# Autodesk Inventor assembly: Assembly1
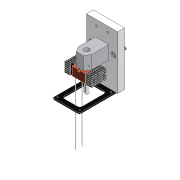
[picture p0: Inventor's stored thumbnail of the model, 180x180]
Saved by Autodesk Inventor 2022.4 (Build 264492000, 492)
## iProperties
Category: -
Company: Universiteit van Amsterdam
Created: 2023-08-21
Part Number: Assembly1
Document SubType Name: Assembly
Designer: RbSrWorkstation1
User Status: Work in Progress
Author: RbSrWorkstation1
Revision Number: A
## Documents named in this file (18)
- D:\VaultLocalWorkingFolder\UvA_MT\Projects\2023\23-0064 Laser diode holder Prem\20_3D-Models\23-0064  Laser diode collimator holder.iam
- D:\VaultLocalWorkingFolder\UvA_MT\Projects\2023\23-0064 Laser diode holder Prem\20_3D-Models\K+S 20C-A4.5-07.ipt
- D:\VaultLocalWorkingFolder\UvA_MT\Projects\2023\23-0064 Laser diode holder Prem\20_3D-Models\23-0064 Diode holder.ipt
- D:\VaultLocalWorkingFolder\UvA_MT\Projects\2023\23-0064 Laser diode holder Prem\20_3D-Models\23-0064 Cooling block.ipt
- D:\VaultLocalWorkingFolder\UvA_MT\Projects\2023\23-0064 Laser diode holder Prem\20_3D-Models\TECF1S.ipt
- D:\VaultLocalWorkingFolder\UvA_MT\Projects\2023\23-0064 Laser diode holder Prem\20_3D-Models\ick_bga_33x33x14.ipt
- D:\VaultLocalWorkingFolder\UvA_MT\Projects\2023\23-0064 Laser diode holder Prem\20_3D-Models\23-0064 Base plate.ipt
- D:\VaultLocalWorkingFolder\UvA_MT\Projects\2023\23-0064 Laser diode holder Prem\20_3D-Models\23-0064  PCB plate.ipt
- D:\VaultLocalWorkingFolder\UvA_MT\Content_Center_Files\en-US\DIN 912\DIN 912 - M5 x 0.8 x 10 x 8.ipt
- D:\VaultLocalWorkingFolder\UvA_MT\Content_Center_Files\en-US\DIN 912\DIN 912 - M6 x 1 x 20 x 17.5.ipt
- D:\VaultLocalWorkingFolder\UvA_MT\Content_Center_Files\en-US\DIN 912\DIN 912 - M3 x 0.5 x 20 x 18.75.ipt
- D:\VaultLocalWorkingFolder\UvA_MT\Content_Center_Files\en-US\DIN 912\DIN 912 - M2.5 x 0.45 x 16 x 14.875.ipt
- D:\VaultLocalWorkingFolder\UvA_MT\Content_Center_Files\en-US\DIN 913\DIN 913 - M2.5 x 3.ipt
- D:\VaultLocalWorkingFolder\UvA_MT\Content_Center_Files\en-US\DIN 912\DIN 912 - M3 x 0.5 x 10 x 8.75.ipt
- D:\VaultLocalWorkingFolder\UvA_MT\Content_Center_Files\en-US\DIN 912\DIN 912 - M5 x 0.8 x 16 x 14.ipt
- D:\VaultLocalWorkingFolder\UvA_MT\Content_Center_Files\en-US\DIN ISO 8734(1A)\ISO 8734 - 4 x 16 - ADIN EN (1).ipt
- D:\VaultLocalWorkingFolder\UvA_MT\Content_Center_Files\en-US\DIN 912\DIN 912 - M3 x 0.5 x 6 x 4.75.ipt
- D:\VaultLocalWorkingFolder\UvA_MT\Projects\2023\23-0064 Laser diode holder Prem\20_3D-Models\23-0064 Adjustment tool.ipt
## Components (28 placed, 17 different names)
1. 23-0064 Diode holder:1 — Mate:16, Mate:17, Angle:2, Mate:23, Mate:24, Mate:25
2. 23-0064 Cooling block:1 — Mate:13, Angle:1, Mate:14, Mate:15, Angle:2, Mate:19, Mate:21, Mate:22, Insert:5, Insert:6, Insert:7, Insert:8, Flush:11, Mate:27, Mate:28, Flush:14, Flush:15, Mate:31
3. 23-0064 Base plate:1 — Mate:23, Mate:24, Mate:25, Mate:26, Flush:8, Flush:9, Insert:3, Insert:4, Insert:15, Insert:16, Mate:29, Mate:30, Flush:12
4. 23-0064  PCB plate:1 — Mate:26, Flush:8, Flush:9, Insert:1, Insert:2
5. K+S 20C-A4.5-07:1 — Mate:13, Angle:1, Mate:14, Mate:16, Mate:17
6. TECF1S:1 — Mate:15, Mate:18, Flush:14, Flush:15
7. ick_bga_33x33x14:1 — Mate:19, Flush:7, Mate:22, Insert:12, Insert:14
8. ick_bga_33x33x14:2 — Mate:18, Mate:20, Flush:7, Mate:21, Insert:9, Insert:10, Insert:11
9. 23-0064 Adjustment tool:1 — Mate:31
10. DIN 912 - replaced by DIN EN ISO 4762 M5 x 10:1 — Insert:1
11. DIN 912 - replaced by DIN EN ISO 4762 M5 x 10:2 — Insert:2
12. DIN 912 - replaced by DIN EN ISO 4762 M6 x 20:1 — Insert:3
13. DIN 912 - replaced by DIN EN ISO 4762 M6 x 20:2 — Insert:4
14. DIN 912 - replaced by DIN EN ISO 4762 M3 x 20:1 — Insert:5
15. DIN 912 - replaced by DIN EN ISO 4762 M3 x 20:2 — Insert:6
16. DIN 912 - replaced by DIN EN ISO 4762 M2,5 x 16:1 — Insert:7
17. DIN 912 - replaced by DIN EN ISO 4762 M2,5 x 16:2 — Insert:8
18. DIN 913 M2.5 x 3:1 — Flush:10, Flush:11, Mate:28
19. DIN 913 M2.5 x 3:2 — Flush:10, Mate:27
20. DIN 912 - replaced by DIN EN ISO 4762 M3 x 10:6 — Insert:9
21. DIN 912 - replaced by DIN EN ISO 4762 M3 x 10:5 — Insert:10
22. DIN 912 - replaced by DIN EN ISO 4762 M3 x 10:1 — Insert:11
23. DIN 912 - replaced by DIN EN ISO 4762 M3 x 6:1 — Insert:12
24. DIN 912 - replaced by DIN EN ISO 4762 M3 x 6:2 — Insert:14
25. DIN 912 - replaced by DIN EN ISO 4762 M5 x 16:1 — Insert:15
26. DIN 912 - replaced by DIN EN ISO 4762 M5 x 16:2 — Insert:16
27. DIN EN 28734 A - replaced by DIN EN ISO 8734 4 x 16 - A:1 — Mate:29, Flush:12, Flush:13
28. DIN EN 28734 A - replaced by DIN EN ISO 8734 4 x 16 - A:2 — Mate:30, Flush:13
## Relationships (45: Mate 19, Insert 15, Flush 9, Angle 2)
- Mate:13: 23-0064 Cooling block:1 ↔ K+S 20C-A4.5-07:1
- Angle:1 (0 deg): 23-0064 Cooling block:1 ↔ K+S 20C-A4.5-07:1
- Mate:14: 23-0064 Cooling block:1 ↔ K+S 20C-A4.5-07:1
- Mate:15: 23-0064 Cooling block:1 ↔ TECF1S:1
- Mate:16: 23-0064 Diode holder:1 ↔ K+S 20C-A4.5-07:1
- Mate:17: 23-0064 Diode holder:1 ↔ K+S 20C-A4.5-07:1
- Angle:2 (0 deg): 23-0064 Diode holder:1 ↔ 23-0064 Cooling block:1
- Mate:18: TECF1S:1 ↔ ick_bga_33x33x14:2
- Mate:19: 23-0064 Cooling block:1 ↔ ick_bga_33x33x14:1
- Mate:20 (-16.5 mm): ick_bga_33x33x14:2
- Flush:7: ick_bga_33x33x14:1 ↔ ick_bga_33x33x14:2
- Mate:21: 23-0064 Cooling block:1 ↔ ick_bga_33x33x14:2
- Mate:22: 23-0064 Cooling block:1 ↔ ick_bga_33x33x14:1
- Mate:23: 23-0064 Diode holder:1 ↔ 23-0064 Base plate:1
- Mate:24: 23-0064 Diode holder:1 ↔ 23-0064 Base plate:1
- Mate:25: 23-0064 Diode holder:1 ↔ 23-0064 Base plate:1
- Mate:26: 23-0064 Base plate:1 ↔ 23-0064  PCB plate:1
- Flush:8 (2 mm): 23-0064 Base plate:1 ↔ 23-0064  PCB plate:1
- Flush:9 (5 mm): 23-0064 Base plate:1 ↔ 23-0064  PCB plate:1
- Insert:1: 23-0064  PCB plate:1 ↔ DIN 912 - replaced by DIN EN ISO 4762 M5 x 10:1
- Insert:2: 23-0064  PCB plate:1 ↔ DIN 912 - replaced by DIN EN ISO 4762 M5 x 10:2
- Insert:3: 23-0064 Base plate:1 ↔ DIN 912 - replaced by DIN EN ISO 4762 M6 x 20:1
- Insert:4: 23-0064 Base plate:1 ↔ DIN 912 - replaced by DIN EN ISO 4762 M6 x 20:2
- Insert:5: 23-0064 Cooling block:1 ↔ DIN 912 - replaced by DIN EN ISO 4762 M3 x 20:1
- Insert:6: 23-0064 Cooling block:1 ↔ DIN 912 - replaced by DIN EN ISO 4762 M3 x 20:2
- Insert:7: 23-0064 Cooling block:1 ↔ DIN 912 - replaced by DIN EN ISO 4762 M2,5 x 16:1
- Insert:8: 23-0064 Cooling block:1 ↔ DIN 912 - replaced by DIN EN ISO 4762 M2,5 x 16:2
- Flush:10: DIN 913 M2.5 x 3:1 ↔ DIN 913 M2.5 x 3:2
- Flush:11: 23-0064 Cooling block:1 ↔ DIN 913 M2.5 x 3:1
- Mate:27: 23-0064 Cooling block:1 ↔ DIN 913 M2.5 x 3:2
- Mate:28: 23-0064 Cooling block:1 ↔ DIN 913 M2.5 x 3:1
- Insert:9: ick_bga_33x33x14:2 ↔ DIN 912 - replaced by DIN EN ISO 4762 M3 x 10:6
- Insert:10: ick_bga_33x33x14:2 ↔ DIN 912 - replaced by DIN EN ISO 4762 M3 x 10:5
- Insert:11: ick_bga_33x33x14:2 ↔ DIN 912 - replaced by DIN EN ISO 4762 M3 x 10:1
- Insert:12: ick_bga_33x33x14:1 ↔ DIN 912 - replaced by DIN EN ISO 4762 M3 x 6:1
- Insert:14: ick_bga_33x33x14:1 ↔ DIN 912 - replaced by DIN EN ISO 4762 M3 x 6:2
- Insert:15: 23-0064 Base plate:1 ↔ DIN 912 - replaced by DIN EN ISO 4762 M5 x 16:1
- Insert:16: 23-0064 Base plate:1 ↔ DIN 912 - replaced by DIN EN ISO 4762 M5 x 16:2
- Mate:29: 23-0064 Base plate:1 ↔ DIN EN 28734 A - replaced by DIN EN ISO 8734 4 x 16 - A:1
- Mate:30: 23-0064 Base plate:1 ↔ DIN EN 28734 A - replaced by DIN EN ISO 8734 4 x 16 - A:2
- Flush:12 (8 mm): 23-0064 Base plate:1 ↔ DIN EN 28734 A - replaced by DIN EN ISO 8734 4 x 16 - A:1
- Flush:13: DIN EN 28734 A - replaced by DIN EN ISO 8734 4 x 16 - A:1 ↔ DIN EN 28734 A - replaced by DIN EN ISO 8734 4 x 16 - A:2
- Flush:14 (8.5 mm): 23-0064 Cooling block:1 ↔ TECF1S:1
- Flush:15 (1 mm): 23-0064 Cooling block:1 ↔ TECF1S:1
- Mate:31: 23-0064 Cooling block:1 ↔ 23-0064 Adjustment tool:1
